# Autodesk Inventor assembly: ClampHorn
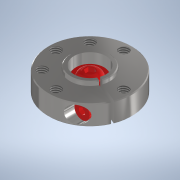
[picture p0: Inventor's stored thumbnail of the model, 180x180]
Saved by Autodesk Inventor 2020 (Build 240168000, 168)
## iProperties
Created: 2022-03-18
Part Number: ClampHorn
Document SubType Name: Assembly
Designer: MasatoKubotera
Author: MasatoKubotera
## Documents named in this file (4)
- C:\Users\MasatoKubotera\Documents\Inventor\SUSTAINA-OP\ReadyMade\KONDO\ClampHorn.iam
- C:\Users\MasatoKubotera\Documents\Inventor\SUSTAINA-OP\ReadyMade\KONDO\ClampHorn.ipt
- C:\Users\MasatoKubotera\Documents\Inventor\SUSTAINA-OP\ReadyMade\Screw\CSH-STH-M2-12.ipt
- C:\Users\MasatoKubotera\Documents\Inventor\SUSTAINA-OP\ReadyMade\Screw\620103008.ipt
## Components (3 placed, 3 different names)
1. ClampHorn:1 — メイト:1, メイト:2, メイト:3, 挿入:1, 挿入:2
2. CSH-STH-M2-12:1 — 挿入:1
3. 620103008:1 — 挿入:2
## Relationships (5: Mate 3, Insert 2)
- メイト:1 [Mate]: ClampHorn:1
- メイト:2 [Mate]: ClampHorn:1
- メイト:3 [Mate]: ClampHorn:1
- 挿入:1 [Insert]: ClampHorn:1 ↔ CSH-STH-M2-12:1
- 挿入:2 [Insert]: ClampHorn:1 ↔ 620103008:1
